# Autodesk Inventor assembly: Assemblage carte_ecran
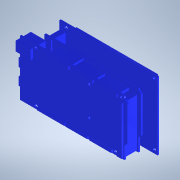
[picture p0: Inventor's stored thumbnail of the model, 180x180]
Saved by Autodesk Inventor 2020 (Build 240168000, 168)
## iProperties
Created: 2020-01-01
Part Number: Assemblage carte_ecran
Document SubType Name: Assembly
Designer: Manuel Enzo
Author: Manuel Enzo
## Documents named in this file (4)
- C:\Users\enzom\Desktop\Projet arduino\Modélisation\Assemblage carte_ecran.iam
- C:\Users\enzom\Desktop\Projet arduino\Modélisation\Adaptateur écran_carte.ipt
- C:\Users\enzom\Desktop\Projet arduino\Modélisation\Carte Due.ipt
- C:\Users\enzom\Desktop\Projet arduino\Modélisation\Ecran.ipt
## Components (3 placed, 3 different names)
1. Carte Due:1 — Placage:2, Affleurement:3, Affleurement:4
2. Ecran:1 — Placage:1, Affleurement:1, Affleurement:2
3. Adaptateur écran_carte:2 — Placage:1, Affleurement:1, Affleurement:2, Placage:2, Affleurement:3, Affleurement:4
## Relationships (6: Flush 4, Mate 2)
- Placage:1 [Mate]: Ecran:1 ↔ Adaptateur écran_carte:2
- Affleurement:1 [Flush]: Ecran:1 ↔ Adaptateur écran_carte:2
- Affleurement:2 [Flush]: Ecran:1 ↔ Adaptateur écran_carte:2
- Placage:2 [Mate]: Carte Due:1 ↔ Adaptateur écran_carte:2
- Affleurement:3 [Flush]: Carte Due:1 ↔ Adaptateur écran_carte:2
- Affleurement:4 [Flush]: Carte Due:1 ↔ Adaptateur écran_carte:2
